# Autodesk Inventor assembly: JibCrane
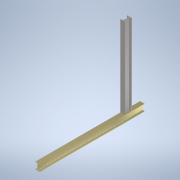
[picture p0: Inventor's stored thumbnail of the model, 180x180]
Saved by Autodesk Inventor 2022 (Build 260153000, 153)
## iProperties
Created: 2023-08-15
Part Number: JibCrane
Document SubType Name: Assembly
Designer: ASUS
Mass: 351146 g
Surface Area: 66689.8 cm^2
Volume: 44732 cm^3
Density: 7.85 g/cm^3
_SolveAssemblyDoc: Frame Generator Solve Assembly
_Version: 15.0.0
Author: ASUS
## Documents named in this file (4)
- C:\Users\ASUS\Documents\Inventor\JibCrane\JibCrane.iam
- C:\Users\ASUS\Documents\Inventor\JibCrane\Columna.ipt
- C:\Users\ASUS\Documents\Inventor\JibCrane\JibCrane\Frame\Columna.iam
- C:\Users\ASUS\Documents\Inventor\JibCrane\Viga-Boceto.ipt
## Components (3 placed, 2 different names)
1. Columna:1
2. Columna:2 [sub-assembly] — Nivelación:1
3. Viga-Boceto:1 — Nivelación:1
## Relationships (1: Flush 1)
- Nivelación:1 [Flush]: Columna:2 ↔ Viga-Boceto:1
## Named parameters: Log_Col = 4749.8 mm, Log_Bra = 50.8 mm, Log_Viga = 1 mm, CD = 2540 mm, BC = 1473.2 mm, AB = 736.6 mm, BE = 1473.2 mm, EF0 = 2184.4 mm
